# Autodesk Inventor assembly: Placed cabinet for drawers
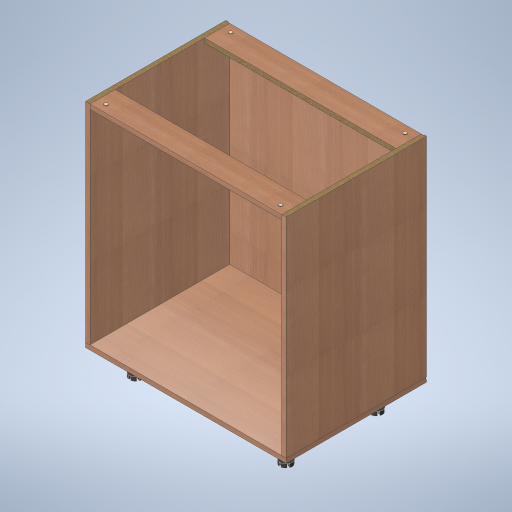
[picture p0: Inventor's stored thumbnail of the model, 512x512]
Saved by Autodesk Inventor 2024 (Build 280153000, 153)
## iProperties
RuleStatus: InUse
Created: 2017-02-01
Part Number: Placed cabinet for drawers
Document SubType Name: Assembly
Designer: SvetlanaB
Description: Placed cabinet for drawers
Author: SvetlanaB
## Documents named in this file (17)
- C:\W4INV 2024 Design\iBOX LIBRARY\Kitchen\Standing Cabinets\Cabinet for drawers\Placed cabinet for drawers.iam
- C:\W4INV 2024 Design\iBOX LIBRARY\Kitchen\Standing Cabinets\Cabinet for drawers\Right panel.ipt
- C:\W4INV 2024 Design\iBOX LIBRARY\Kitchen\Standing Cabinets\Cabinet for drawers\Left panel.ipt
- C:\W4INV 2024 Design\iBOX LIBRARY\Kitchen\Standing Cabinets\Cabinet for drawers\Bottom panel.ipt
- C:\W4INV 2024 Design\iBOX LIBRARY\Kitchen\Standing Cabinets\Cabinet for drawers\Back panel.ipt
- C:\W4INV 2024 Design\iBOX LIBRARY\Kitchen\Standing Cabinets\Cabinet for drawers\Top panel.ipt
- C:\W4INV 2024 Design\_LIBRARY\Supports and legs\Legs\ADJUSTABLE LEG\Adjustable leg  BT18.ipt
- C:\W4INV 2024 Design\_LIBRARY\Fixed joints\Confirmat\CONFIRMAT\Confirmat L50 NB T18 PB T 18.ipt
- C:\W4INV 2024 Design\iBOX LIBRARY\Kitchen\Standing Cabinets\Cabinet for drawers\Placed cabinet for drawers.ipt
- C:\W4INV 2024 Design\_LIBRARY\Fixed joints\Minifix joint\MINIFIX D15 v2\Minifix D15 & Dowel L34 & Cap D15 PB T18 LH.ipt
- C:\W4INV 2024 Design\_LIBRARY\Fixed joints\Minifix joint\MINIFIX D15 v2\Minifix D15 & Dowel L34 & Cap D15 PB T18 RH.ipt
- C:\W4INV 2024 Design\_LIBRARY\Fixed joints\Confirmat\CONFIRMAT\Confirmat L50 & Cap D10 NB T18 PB T 18.ipt
- C:\W4INV 2024 Design\iBOX LIBRARY\Kitchen\Standing Cabinets\Cabinet for drawers\Top panel 2.ipt
- C:\W4INV 2024 Design\_LIBRARY\Supports and legs\Legs\ADJUSTABLE LEG\Adjustable leg  BT18 clip included.ipt
- C:\W4INV 2023 Design\LIBRARY\Fixed joints\Confirmat\CONFIRMAT.ipt
- C:\W4INV 2023 Design\LIBRARY\Fixed joints\Minifix joint\MINIFIX D15 v2.ipt
- C:\W4INV 2023 Design\LIBRARY\Supports and legs\Legs\ADJUSTABLE LEG.ipt
## Components (19 placed, 13 different names)
1. @Skeleton
2. Right panel:1 — Pillar Board Side Plane:6, Pillar Board Side Plane:8, Nestled Board Plane:3, Nestled Board Plane:4
3. Left panel:1 — Flush:5, Flush:6, Pillar Board Side Plane:5, Pillar Board Side Plane:7, Nestled Board Plane:1, Nestled Board Plane:2
4. Bottom panel:1 — Flush:1, Flush:2, Flush:3, Flush:4, Bottom board Plane:1, Front (Angle) Plane:1, Bottom board Plane:2, Front (Angle) Plane:2, Bottom board Plane:3, Front (Angle) Plane:3, Bottom board Plane:4, Front (Angle) Plane:4, Nestled Board Plane:5, Nestled Board Plane:6, Nestled Board Plane:7, Nestled Board Plane:8
5. Back panel:1
6. Top panel:1 — Flush:7, Pillar Board Side Plane :4, Pillar Board Side Plane :2
7. Adjustable leg  BT18 clip included:1 — Axis2 Plane:1, Axis Plane:1, Bottom board Plane:1, Front (Angle) Plane:1
8. Adjustable leg  BT18 clip included:2 — Axis2 Plane:2, Axis Plane:2, Bottom board Plane:2, Front (Angle) Plane:2
9. Adjustable leg  BT18:3 — Axis2 Plane:3, Axis Plane:3, Bottom board Plane:3, Front (Angle) Plane:3
10. Adjustable leg  BT18:4 — Axis2 Plane:4, Axis Plane:4, Bottom board Plane:4, Front (Angle) Plane:4
11. Confirmat L50 & Cap D10 NB T18 PB T 18:6 — Axis Plane:9, Pillar Board Side Plane:5, Nestled Board Plane:5
12. Confirmat L50 NB T18 PB T 18:7 — Axis Plane:10, Pillar Board Side Plane:6, Nestled Board Plane:6
13. Confirmat L50 NB T18 PB T 18:8 — Axis Plane:11, Pillar Board Side Plane:7, Nestled Board Plane:7
14. Confirmat L50 NB T18 PB T 18:9 — Axis Plane:12, Pillar Board Side Plane:8, Nestled Board Plane:8
15. Minifix D15 & Dowel L34 & Cap D15 PB T18 LH:1 — Nestled Board Plane:1, Axis Plane:7, Pillar Board Side Plane :1
16. Minifix D15 & Dowel L34 & Cap D15 PB T18 RH:2 — Nestled Board Plane:2, Axis Plane:6, Pillar Board Side Plane :2
17. Minifix D15 & Dowel L34 & Cap D15 PB T18 RH:3 — Nestled Board Plane:3, Axis Plane:5, Pillar Board Side Plane :3
18. Minifix D15 & Dowel L34 & Cap D15 PB T18 LH:4 — Nestled Board Plane:4, Axis Plane:8, Pillar Board Side Plane :4
19. Top panel 2:1 — Flush:31, Pillar Board Side Plane :1, Pillar Board Side Plane :3
## Relationships (48: Mate 28, Flush 16, Angle 4)
- Flush:1 (-100 mm): Bottom panel:1
- Flush:2 (-100 mm): Bottom panel:1
- Flush:3 (-100 mm): Bottom panel:1
- Flush:4 (-100 mm): Bottom panel:1
- Flush:5 (-64 mm): Left panel:1
- Flush:6 (-64 mm): Left panel:1
- Flush:7 (-70 mm): Top panel:1
- Axis2 Plane:1 [Mate]: Adjustable leg  BT18 clip included:1
- Axis Plane:1 [Mate]: Adjustable leg  BT18 clip included:1
- Bottom board Plane:1 [Mate]: Bottom panel:1 ↔ Adjustable leg  BT18 clip included:1
- Front (Angle) Plane:1 [Angle] (0 deg): Bottom panel:1 ↔ Adjustable leg  BT18 clip included:1
- Axis2 Plane:2 [Mate]: Adjustable leg  BT18 clip included:2
- Axis Plane:2 [Mate]: Adjustable leg  BT18 clip included:2
- Bottom board Plane:2 [Mate]: Bottom panel:1 ↔ Adjustable leg  BT18 clip included:2
- Front (Angle) Plane:2 [Angle] (0 deg): Bottom panel:1 ↔ Adjustable leg  BT18 clip included:2
- Axis2 Plane:3 [Mate]: Adjustable leg  BT18:3
- Axis Plane:3 [Mate]: Adjustable leg  BT18:3
- Bottom board Plane:3 [Mate]: Bottom panel:1 ↔ Adjustable leg  BT18:3
- Front (Angle) Plane:3 [Angle] (0 deg): Bottom panel:1 ↔ Adjustable leg  BT18:3
- Axis2 Plane:4 [Mate]: Adjustable leg  BT18:4
- Axis Plane:4 [Mate]: Adjustable leg  BT18:4
- Bottom board Plane:4 [Mate]: Bottom panel:1 ↔ Adjustable leg  BT18:4
- Front (Angle) Plane:4 [Angle] (0 deg): Bottom panel:1 ↔ Adjustable leg  BT18:4
- Axis Plane:9 [Mate]: Confirmat L50 & Cap D10 NB T18 PB T 18:6
- Pillar Board Side Plane:5 [Mate] (-9 mm): Left panel:1 ↔ Confirmat L50 & Cap D10 NB T18 PB T 18:6
- Nestled Board Plane:5 [Flush]: Bottom panel:1 ↔ Confirmat L50 & Cap D10 NB T18 PB T 18:6
- Axis Plane:10 [Mate]: Confirmat L50 NB T18 PB T 18:7
- Pillar Board Side Plane:6 [Mate] (-9 mm): Right panel:1 ↔ Confirmat L50 NB T18 PB T 18:7
- Nestled Board Plane:6 [Flush]: Bottom panel:1 ↔ Confirmat L50 NB T18 PB T 18:7
- Axis Plane:11 [Mate]: Confirmat L50 NB T18 PB T 18:8
- Pillar Board Side Plane:7 [Mate] (-9 mm): Left panel:1 ↔ Confirmat L50 NB T18 PB T 18:8
- Nestled Board Plane:7 [Flush]: Bottom panel:1 ↔ Confirmat L50 NB T18 PB T 18:8
- Axis Plane:12 [Mate]: Confirmat L50 NB T18 PB T 18:9
- Pillar Board Side Plane:8 [Mate] (-9 mm): Right panel:1 ↔ Confirmat L50 NB T18 PB T 18:9
- Nestled Board Plane:8 [Flush]: Bottom panel:1 ↔ Confirmat L50 NB T18 PB T 18:9
- Nestled Board Plane:1 [Mate]: Left panel:1 ↔ Minifix D15 & Dowel L34 & Cap D15 PB T18 LH:1
- Nestled Board Plane:2 [Mate]: Left panel:1 ↔ Minifix D15 & Dowel L34 & Cap D15 PB T18 RH:2
- Axis Plane:6 [Mate]: Minifix D15 & Dowel L34 & Cap D15 PB T18 RH:2
- Nestled Board Plane:3 [Mate]: Right panel:1 ↔ Minifix D15 & Dowel L34 & Cap D15 PB T18 RH:3
- Nestled Board Plane:4 [Mate]: Right panel:1 ↔ Minifix D15 & Dowel L34 & Cap D15 PB T18 LH:4
- Axis Plane:8 [Mate]: Minifix D15 & Dowel L34 & Cap D15 PB T18 LH:4
- Flush:31 (-30 mm): Top panel 2:1
- Axis Plane:5 [Mate]: Minifix D15 & Dowel L34 & Cap D15 PB T18 RH:3
- Axis Plane:7 [Mate]: Minifix D15 & Dowel L34 & Cap D15 PB T18 LH:1
- Pillar Board Side Plane :1 [Flush] (18 mm): Minifix D15 & Dowel L34 & Cap D15 PB T18 LH:1 ↔ Top panel 2:1
- Pillar Board Side Plane :3 [Flush] (18 mm): Minifix D15 & Dowel L34 & Cap D15 PB T18 RH:3 ↔ Top panel 2:1
- Pillar Board Side Plane :4 [Flush] (18 mm): Top panel:1 ↔ Minifix D15 & Dowel L34 & Cap D15 PB T18 LH:4
- Pillar Board Side Plane :2 [Flush] (18 mm): Top panel:1 ↔ Minifix D15 & Dowel L34 & Cap D15 PB T18 RH:2
## Named parameters: Panel_thickness = 18 mm
